# Autodesk Inventor assembly: Fly Wheel Assembly
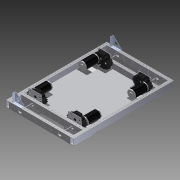
[picture p0: Inventor's stored thumbnail of the model, 180x180]
Saved by Autodesk Inventor 2014 (Build 180170000, 170)
## iProperties
Created: 2014-01-10
Part Number: Fly Wheel Assembly
Document SubType Name: Assembly
Designer: Paul
Author: Paul
## Documents named in this file (18)
- C:\4859cad\Robot\Actual Robot\Fly Wheel\Fly Wheel Assembly.iam
- C:\4859cad\Robot\Structure\Frame Assembly\2x1 Tube 21in.ipt
- C:\4859cad\Robot\Structure\Frame Assembly\2x1 Tube 34in.ipt
- C:\4859cad\Robot\Drivetrain\Drivetrain Assembly\Imported Components\Toughbox-mini\Toughbox-mini_d02.ipt
- C:\4859cad\Robot\Drivetrain\Drivetrain Assembly\Imported Components\Toughbox-mini\Toughbox-mini_d01-5-12.ipt
- C:\4859cad\Robot\KOP STEP\Drive Base Kit\FIRST Drive Base Wide\Parts\Imported Components\CIM Motor SW.ipt\CIM Motor SW.ipt.ipt
- C:\4859cad\Robot\KOP STEP\Drive Base Kit\FIRST Drive Base Wide\Parts\Imported Components\TB Output Shaft Hex L-Base 2.ipt\TB Output Shaft Hex L-Base 2.ipt.ipt
- C:\FRC_CAD\4859cad\Robot\Drivetrain\Imported Components\Hex Versa Hub\Hex Versa Hub.ipt
- C:\FRC_CAD\4859cad\Robot\Drivetrain\Drivetrain Assembly\Imported Components\Right mechanum\Right mechanum.iam
- C:\4859cad\Robot\Structure\Imported Components\T Guesset\T Guesset.ipt
- C:\4859cad\Robot\Structure\Imported Components\L Guesset\L Guesset.ipt
- C:\4859cad\Robot\Structure\Electronics\Belly Board.ipt
- C:\FRC_CAD\4859cad\Robot\Actual Robot\Bumper.ipt
- C:\4859cad\Robot\Structure\Frame Assembly\1x.61 Block 5 in.ipt
- C:\4859cad\Robot\Structure\Frame Assembly\Aluminum Board.ipt
- C:\4859cad\Robot\Structure\Imported Components\Corner Guesset\Corner Guesset.ipt
- CIM Motor SW.ipt
- TB Output Shaft Hex L-Base 2.ipt
## Components (44 placed, 15 different names)
1. Toughbox-mini_d02:1 — Mate:1, Mate:2, Mate:3, Mate:14, Mate:15, Flush:32, Flush:34
2. Toughbox-mini_d01-5-12:1 — Mate:1, Mate:2, Mate:3, Mate:4, Mate:5, Mate:6, Mate:16
3. CIM Motor SW.ipt:1 — Mate:5, Mate:6, Mate:90, Mate:92
4. TB Output Shaft Hex L-Base 2.ipt:1 — Mate:4, Mate:16, Flush:30, Mate:137
5. 2x1 Tube 21in:1 — Mate:7, Flush:1, Flush:2, Mate:8, Flush:3, Flush:4, Mate:13, Flush:12, Flush:15, Mate:102, Mate:134, Flush:48, Mate:136, Mate:137
6. 2x1 Tube 34in:1 — Mate:7, Flush:1, Flush:2, Flush:5, Mate:9, Flush:6, Mate:10, Mate:11, Flush:7, Flush:8, Mate:72, Mate:73, Mate:79, Mate:80, Flush:14, Mate:84, Mate:85, Flush:18, Flush:19, Mate:101, Flush:42
7. 2x1 Tube 21in:2 — Flush:5, Mate:9, Flush:6, Mate:12, Flush:16, Mate:104, Mate:135, Flush:49
8. 2x1 Tube 34in:2 — Mate:8, Flush:3, Flush:4, Mate:75, Mate:76, Mate:81, Mate:82, Mate:83, Flush:13, Mate:86, Flush:17, Mate:89, Mate:103, Mate:114
9. 2x1 Tube 21in:3 — Mate:11, Flush:7, Mate:13, Mate:14, Mate:15, Mate:24, Mate:25, Mate:88, Mate:111, Mate:112, Flush:33, Flush:37, Flush:43
10. 2x1 Tube 21in:4 — Mate:10, Flush:8, Mate:12, Mate:34, Mate:35, Mate:43, Mate:50, Mate:113, Flush:35, Flush:40, Flush:41
11. Toughbox-mini_d02:2 — Mate:24, Mate:25, Flush:38
12. Toughbox-mini_d01-5-12:2 — Mate:26
13. CIM Motor SW.ipt:2 — Mate:26
14. TB Output Shaft Hex L-Base 2.ipt:2 — Mate:136
15. Toughbox-mini_d02:3 — Mate:34, Mate:35, Flush:39
16. Toughbox-mini_d01-5-12:3
17. CIM Motor SW.ipt:3
18. TB Output Shaft Hex L-Base 2.ipt:3 — Mate:53, Mate:54
19. Toughbox-mini_d02:4 — Mate:43, Flush:32, Flush:36
20. Toughbox-mini_d01-5-12:4 — Mate:55
21. CIM Motor SW.ipt:4 — Mate:55, Mate:90, Mate:92
22. TB Output Shaft Hex L-Base 2.ipt:4 — Mate:48, Mate:49
23. Hex Versa Hub:1 — Mate:46, Mate:47, Rotation:1, Mate:48, Mate:49
24. Hex Versa Hub:2 — Mate:51, Mate:52, Mate:53, Mate:54
25. Right mechanum:1 [sub-assembly] — Mate:51, Mate:52
26. Right mechanum:2 [sub-assembly] — Mate:46, Mate:47, Rotation:1, Mate:50
27. T Guesset:5 — Mate:72, Mate:73, Mate:113, Mate:118
28. T Guesset:6 — Mate:79, Mate:80, Mate:112, Mate:117
29. T Guesset:7 — Mate:75, Mate:76, Mate:114, Mate:116
30. T Guesset:8 — Mate:81, Mate:82, Mate:111, Mate:115
31. L Guesset:1 — Flush:14, Flush:15, Mate:84
32. L Guesset:2 — Mate:83, Flush:12, Flush:13
33. L Guesset:3 — Mate:85, Flush:18, Flush:19
34. L Guesset:4 — Mate:86, Flush:16, Flush:17
35. Belly Board:1 — Mate:88, Mate:89, Flush:41, Mate:119
36. Bumper:1 — Mate:101, Mate:102, Flush:30, Flush:31
37. Bumper:2 — Mate:103, Mate:104, Flush:31
38. 1x.61 Block 5 in:1 — Mate:115, Flush:33, Flush:34
39. 1x.61 Block 5 in:2 — Mate:116, Flush:35, Flush:36
40. 1x.61 Block 5 in:3 — Mate:117, Flush:37, Flush:38
41. 1x.61 Block 5 in:4 — Mate:118, Flush:39, Flush:40
42. Aluminum Board:1 — Mate:119, Flush:42, Flush:43
43. Corner Guesset:1 — Mate:134, Flush:48
44. Corner Guesset:2 — Mate:135, Flush:49
## Relationships (117: Mate 84, Flush 32, RelateRotation 1)
- Mate:1: Toughbox-mini_d02:1 ↔ Toughbox-mini_d01-5-12:1
- Mate:2: Toughbox-mini_d02:1 ↔ Toughbox-mini_d01-5-12:1
- Mate:3: Toughbox-mini_d02:1 ↔ Toughbox-mini_d01-5-12:1
- Mate:4: Toughbox-mini_d01-5-12:1 ↔ TB Output Shaft Hex L-Base 2.ipt:1
- Mate:5: Toughbox-mini_d01-5-12:1 ↔ CIM Motor SW.ipt:1
- Mate:6: Toughbox-mini_d01-5-12:1 ↔ CIM Motor SW.ipt:1
- Mate:7: 2x1 Tube 21in:1 ↔ 2x1 Tube 34in:1
- Flush:1: 2x1 Tube 21in:1 ↔ 2x1 Tube 34in:1
- Flush:2: 2x1 Tube 21in:1 ↔ 2x1 Tube 34in:1
- Mate:8: 2x1 Tube 21in:1 ↔ 2x1 Tube 34in:2
- Flush:3: 2x1 Tube 21in:1 ↔ 2x1 Tube 34in:2
- Flush:4: 2x1 Tube 21in:1 ↔ 2x1 Tube 34in:2
- Flush:5: 2x1 Tube 34in:1 ↔ 2x1 Tube 21in:2
- Mate:9: 2x1 Tube 34in:1 ↔ 2x1 Tube 21in:2
- Flush:6: 2x1 Tube 34in:1 ↔ 2x1 Tube 21in:2
- Mate:10: 2x1 Tube 34in:1 ↔ 2x1 Tube 21in:4
- Mate:11: 2x1 Tube 34in:1 ↔ 2x1 Tube 21in:3
- Flush:7: 2x1 Tube 34in:1 ↔ 2x1 Tube 21in:3
- Flush:8: 2x1 Tube 34in:1 ↔ 2x1 Tube 21in:4
- Mate:12 (76.2 mm): 2x1 Tube 21in:2 ↔ 2x1 Tube 21in:4
- Mate:13 (76.2 mm): 2x1 Tube 21in:1 ↔ 2x1 Tube 21in:3
- Mate:14 (15.748 mm): Toughbox-mini_d02:1 ↔ 2x1 Tube 21in:3
- Mate:15: Toughbox-mini_d02:1 ↔ 2x1 Tube 21in:3
- Mate:16: Toughbox-mini_d01-5-12:1 ↔ TB Output Shaft Hex L-Base 2.ipt:1
- [Mate]: Toughbox-mini_d02:2 ↔ Toughbox-mini_d01-5-12:2
- [Mate]: Toughbox-mini_d02:2 ↔ Toughbox-mini_d01-5-12:2
- [Mate]: Toughbox-mini_d02:2 ↔ Toughbox-mini_d01-5-12:2
- [Mate]: Toughbox-mini_d01-5-12:2 ↔ TB Output Shaft Hex L-Base 2.ipt:2
- [Mate]: Toughbox-mini_d01-5-12:2 ↔ CIM Motor SW.ipt:2
- [Mate]: Toughbox-mini_d01-5-12:2 ↔ TB Output Shaft Hex L-Base 2.ipt:2
- Mate:24: 2x1 Tube 21in:3 ↔ Toughbox-mini_d02:2
- Mate:25 (15.748 mm): 2x1 Tube 21in:3 ↔ Toughbox-mini_d02:2
- Mate:26: Toughbox-mini_d01-5-12:2 ↔ CIM Motor SW.ipt:2
- [Mate]: Toughbox-mini_d02:3 ↔ Toughbox-mini_d01-5-12:3
- [Mate]: Toughbox-mini_d02:3 ↔ Toughbox-mini_d01-5-12:3
- [Mate]: Toughbox-mini_d02:3 ↔ Toughbox-mini_d01-5-12:3
- [Mate]: Toughbox-mini_d01-5-12:3 ↔ TB Output Shaft Hex L-Base 2.ipt:3
- [Mate]: Toughbox-mini_d01-5-12:3 ↔ CIM Motor SW.ipt:3
- [Mate]: Toughbox-mini_d01-5-12:3 ↔ CIM Motor SW.ipt:3
- [Mate]: Toughbox-mini_d01-5-12:3 ↔ TB Output Shaft Hex L-Base 2.ipt:3
- Mate:34 (15.748 mm): 2x1 Tube 21in:4 ↔ Toughbox-mini_d02:3
- Mate:35: 2x1 Tube 21in:4 ↔ Toughbox-mini_d02:3
- [Mate]: Toughbox-mini_d02:4 ↔ Toughbox-mini_d01-5-12:4
- [Mate]: Toughbox-mini_d02:4 ↔ Toughbox-mini_d01-5-12:4
- [Mate]: Toughbox-mini_d02:4 ↔ Toughbox-mini_d01-5-12:4
- [Mate]: Toughbox-mini_d01-5-12:4 ↔ TB Output Shaft Hex L-Base 2.ipt:4
- [Mate]: Toughbox-mini_d01-5-12:4 ↔ CIM Motor SW.ipt:4
- [Mate]: Toughbox-mini_d01-5-12:4 ↔ TB Output Shaft Hex L-Base 2.ipt:4
- Mate:43: 2x1 Tube 21in:4 ↔ Toughbox-mini_d02:4
- Mate:46: Hex Versa Hub:1 ↔ Right mechanum:2
- Mate:47: Hex Versa Hub:1 ↔ Right mechanum:2
- Rotation:1 [RelateRotation] (1 ul): Hex Versa Hub:1 ↔ Right mechanum:2
- Mate:48: TB Output Shaft Hex L-Base 2.ipt:4 ↔ Hex Versa Hub:1
- Mate:49: TB Output Shaft Hex L-Base 2.ipt:4 ↔ Hex Versa Hub:1
- Mate:50 (16.51 mm): 2x1 Tube 21in:4 ↔ Right mechanum:2
- Mate:51: Hex Versa Hub:2 ↔ Right mechanum:1
- Mate:52: Hex Versa Hub:2 ↔ Right mechanum:1
- Mate:53: TB Output Shaft Hex L-Base 2.ipt:3 ↔ Hex Versa Hub:2
- Mate:54: TB Output Shaft Hex L-Base 2.ipt:3 ↔ Hex Versa Hub:2
- Mate:55: Toughbox-mini_d01-5-12:4 ↔ CIM Motor SW.ipt:4
- Mate:72: 2x1 Tube 34in:1 ↔ T Guesset:5
- Mate:73: 2x1 Tube 34in:1 ↔ T Guesset:5
- Mate:75: 2x1 Tube 34in:2 ↔ T Guesset:7
- Mate:76: 2x1 Tube 34in:2 ↔ T Guesset:7
- Mate:79: 2x1 Tube 34in:1 ↔ T Guesset:6
- Mate:80: 2x1 Tube 34in:1 ↔ T Guesset:6
- Mate:81: 2x1 Tube 34in:2 ↔ T Guesset:8
- Mate:82: 2x1 Tube 34in:2 ↔ T Guesset:8
- Mate:83: 2x1 Tube 34in:2 ↔ L Guesset:2
- Flush:12: 2x1 Tube 21in:1 ↔ L Guesset:2
- Flush:13: 2x1 Tube 34in:2 ↔ L Guesset:2
- Flush:14: 2x1 Tube 34in:1 ↔ L Guesset:1
- Flush:15: 2x1 Tube 21in:1 ↔ L Guesset:1
- Mate:84: 2x1 Tube 34in:1 ↔ L Guesset:1
- Mate:85: 2x1 Tube 34in:1 ↔ L Guesset:3
- Mate:86: 2x1 Tube 34in:2 ↔ L Guesset:4
- Flush:16: 2x1 Tube 21in:2 ↔ L Guesset:4
- Flush:17: 2x1 Tube 34in:2 ↔ L Guesset:4
- Flush:18: 2x1 Tube 34in:1 ↔ L Guesset:3
- Flush:19: 2x1 Tube 34in:1 ↔ L Guesset:3
- Mate:88: 2x1 Tube 21in:3 ↔ Belly Board:1
- Mate:89: 2x1 Tube 34in:2 ↔ Belly Board:1
- Mate:90: CIM Motor SW.ipt:1 ↔ CIM Motor SW.ipt:4
- Mate:92: CIM Motor SW.ipt:1 ↔ CIM Motor SW.ipt:4
- Mate:101: 2x1 Tube 34in:1 ↔ Bumper:1
- Mate:102: 2x1 Tube 21in:1 ↔ Bumper:1
- Mate:103: 2x1 Tube 34in:2 ↔ Bumper:2
- Mate:104: 2x1 Tube 21in:2 ↔ Bumper:2
- Flush:30 (19.05 mm): TB Output Shaft Hex L-Base 2.ipt:1 ↔ Bumper:1
- Flush:31: Bumper:1 ↔ Bumper:2
- Mate:111: 2x1 Tube 21in:3 ↔ T Guesset:8
- Mate:112: 2x1 Tube 21in:3 ↔ T Guesset:6
- Mate:113: 2x1 Tube 21in:4 ↔ T Guesset:5
- Mate:114: 2x1 Tube 34in:2 ↔ T Guesset:7
- Flush:32: Toughbox-mini_d02:1 ↔ Toughbox-mini_d02:4
- Mate:115: T Guesset:8 ↔ 1x.61 Block 5 in:1
- Flush:33: 2x1 Tube 21in:3 ↔ 1x.61 Block 5 in:1
- Flush:34: Toughbox-mini_d02:1 ↔ 1x.61 Block 5 in:1
- Mate:116: T Guesset:7 ↔ 1x.61 Block 5 in:2
- Flush:35: 2x1 Tube 21in:4 ↔ 1x.61 Block 5 in:2
- Flush:36: Toughbox-mini_d02:4 ↔ 1x.61 Block 5 in:2
- Mate:117: T Guesset:6 ↔ 1x.61 Block 5 in:3
- Flush:37: 2x1 Tube 21in:3 ↔ 1x.61 Block 5 in:3
- Flush:38: Toughbox-mini_d02:2 ↔ 1x.61 Block 5 in:3
- Mate:118: T Guesset:5 ↔ 1x.61 Block 5 in:4
- Flush:39: Toughbox-mini_d02:3 ↔ 1x.61 Block 5 in:4
- Flush:40: 2x1 Tube 21in:4 ↔ 1x.61 Block 5 in:4
- Flush:41: 2x1 Tube 21in:4 ↔ Belly Board:1
- Mate:119: Belly Board:1 ↔ Aluminum Board:1
- Flush:42: 2x1 Tube 34in:1 ↔ Aluminum Board:1
- Flush:43: 2x1 Tube 21in:3 ↔ Aluminum Board:1
- Mate:134: 2x1 Tube 21in:1 ↔ Corner Guesset:1
- Flush:48: 2x1 Tube 21in:1 ↔ Corner Guesset:1
- Mate:135: 2x1 Tube 21in:2 ↔ Corner Guesset:2
- Flush:49: 2x1 Tube 21in:2 ↔ Corner Guesset:2
- Mate:136: 2x1 Tube 21in:1 ↔ TB Output Shaft Hex L-Base 2.ipt:2
- Mate:137: TB Output Shaft Hex L-Base 2.ipt:1 ↔ 2x1 Tube 21in:1
## Named parameters: d124_d123 = 0 mm, d125_d99 = 0 mm, d126_d100 = 0 mm, d127_d101 = 0 mm, d128_d102 = 0 mm, d130_d104 = 0 mm, d134_d123 = 0 mm, d135_d99 = 0 mm, d136_d100 = 0 mm, d137_d101 = 0 mm, d138_d102 = 0 mm, d139_d103 = 0 mm, d140_d104 = 0 mm, d143_d123 = 0 mm, d144_d99 = 0 mm, d145_d100 = 0 mm, d146_d101 = 0 mm, d147_d102 = 0 mm, d149_d104 = 0 mm
